# Autodesk Inventor assembly: Drive Roller Assembly 2
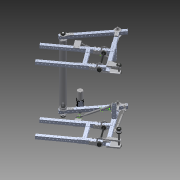
[picture p0: Inventor's stored thumbnail of the model, 180x180]
Saved by Autodesk Inventor 2014 (Build 180170000, 170)
## iProperties
Created: 2014-01-12
Part Number: Drive Roller Assembly 2
Document SubType Name: Assembly
Designer: Michael
Mass: 4835.9 g
Surface Area: 14934.6 cm^2
Volume: 1370.56 cm^3
Density: 3.52842 g/cm^3
Author: Michael
## Documents named in this file (35)
- C:\Users\Michael\Documents\GitHub\2014buildCAD\New Collector\Drive Roller Assembly 2.iam
- C:\Users\Michael\Documents\GitHub\2014buildCAD\Collector\Hex Shaft Collar 1-2 in (7552K500).ipt
- C:\Users\Michael\Documents\GitHub\2014buildCAD\Collector\Roller End Cap Drive (3-D Printed).ipt
- C:\Users\Michael\Documents\GitHub\2014buildCAD\Collector\Vex Pro VersaPlanetary Side Mount.ipt
- C:\Users\Michael\Documents\GitHub\2014buildCAD\Collector\VersaPlanetary (Fixed).iam
- C:\Users\Michael\Documents\GitHub\2014buildCAD\New Collector\Polycarbonate Roller 2 OD 1-16 Thick (8585K64).ipt
- C:\Users\Michael\Documents\GitHub\2014buildCAD\New Collector\Hex Bearing 1-2 in (FR8ZZ-Hex, am-0279).ipt
- C:\Users\Michael\Documents\GitHub\2014buildCAD\New Collector\Hex Shaft Collar 1-2 in (7552K500).ipt
- C:\Users\Michael\Documents\GitHub\2014buildCAD\New Collector\Roller End Cap Drive (3-D Printed).ipt
- C:\Users\Michael\Documents\GitHub\2014buildCAD\New Collector\Vex Pro End Bearing Mount.ipt
- C:\Users\Michael\Documents\GitHub\2014buildCAD\New Collector\Vex Pro 1x1 rectangular tubing 14 in length.ipt
- C:\Users\Michael\Documents\GitHub\2014buildCAD\New Collector\Hex Shaft Aluminum 1-2 in (am-2291).ipt
- C:\Users\Michael\Documents\GitHub\2014buildCAD\New Collector\Timing Pulley (HTD 5mm) - 18T 9mm Double Flange, 1-2 in Hex (VexPro).ipt
- C:\Users\Michael\Documents\GitHub\2014buildCAD\New Collector\Clamp with Piston Assembly.iam
- C:\Users\Michael\Documents\GitHub\2014buildCAD\New Collector\Vex Pro 90 degree gusset.ipt
- C:\Users\Michael\Documents\GitHub\2014buildCAD\New Collector\Vex Pro 1x1 rectangular tubing 2 in length.ipt
- C:\Users\Michael\Documents\GitHub\2014buildCAD\New Collector\Hex Shaft 3-8 in (am-0855).ipt
- C:\Users\Michael\Documents\GitHub\2014buildCAD\New Collector\Hex Shaft Collar 3-8 in (7552K300).ipt
- C:\Users\Michael\Documents\GitHub\2014buildCAD\New Collector\3 Postion Pneumatic Cylinder (9-16 in Bore, .25 in,2 in stroke).iam
- C:\Users\Michael\Documents\GitHub\2014buildCAD\New Collector\Hex Shaft 1-2 in (am-0856).ipt
- C:\Users\Michael\Documents\GitHub\2014buildCAD\New Collector\Spacer 2.ipt
- C:\Users\Michael\Documents\GitHub\2014buildCAD\New Collector\Gusset 3 (R-R) (Custom) ipt.ipt
- C:\Users\Michael\Documents\GitHub\2014buildCAD\New Collector\Gusset 3 (L-R) (Custom).ipt
- C:\Users\Michael\Documents\GitHub\2014buildCAD\New Collector\Gusset 3 (L-L) (Custom) ipt.ipt
- C:\Users\Michael\Documents\GitHub\2014buildCAD\New Collector\Gusset 3 (R-L) (Custom).ipt
- C:\Users\Michael\Documents\GitHub\2014buildCAD\New Collector\Vex Pro 1x1 rectangular tubing 4 in length.ipt
- C:\Users\Michael\Documents\GitHub\2014buildCAD\New Collector\Pneumatic Piston Front Flange (Lt Custom).ipt
- C:\Users\Michael\Documents\GitHub\2014buildCAD\New Collector\Pneumatic Piston Front Flange (Rt Custom).ipt
- C:\Users\Michael\Documents\GitHub\2014buildCAD\New Collector\Pneumatic Piston Back Flange (Rt Custom).ipt
- C:\Users\Michael\Documents\GitHub\2014buildCAD\New Collector\Bearing Mount Spacer 1-8 in.ipt
- C:\Users\Michael\Documents\GitHub\2014buildCAD\New Collector\Vex Pro 1x1 rectangular tubing 14 in length (roller).ipt
- C:\Users\Michael\Documents\GitHub\2014buildCAD\New Collector\Pneumatic Piston Back Flange (Right Custom).ipt
- C:\Users\Michael\Documents\GitHub\2014buildCAD\New Collector\Hex Shaft 1-2 in 5 in long (am-0856).ipt
- C:\Users\Michael\Documents\GitHub\2014buildCAD\New Collector\Vex Pro End Bearing Mount (Bolt).ipt
- C:\Users\Michael\Documents\GitHub\2014buildCAD\New Collector\Roller Piston (3 Position, .25 and 1.125 in stroke, 9-16 bore).iam
## Components (96 placed, 32 different names)
1. Roller End Cap Drive (3-D Printed):2 — Mate:154, Mate:155, Mate:157, Mate:158, Mate:466, Mate:469
2. Vex Pro VersaPlanetary Side Mount:1 — Insert:29, Insert:30, Mate:566, Mate:779, Mate:780
3. VersaPlanetary (Fixed):1 [sub-assembly] — Insert:29, Insert:30, Mate:113, Mate:114, Mate:120, Mate:121, Mate:153
4. Hex Shaft Collar 1-2 in (7552K500):9 — Mate:113, Mate:114
5. Hex Shaft Collar 1-2 in (7552K500):10 — Mate:120, Mate:121
6. Polycarbonate Roller 2 OD 1-16 Thick (8585K64):3 — Mate:157, Mate:158, Mate:159, Mate:160
7. Hex Bearing 1-2 in (FR8ZZ-Hex, am-0279):3 — Mate:128, Mate:129, Mate:134, Mate:466
8. Roller End Cap Drive (3-D Printed):5 — Mate:159, Mate:160, Mate:632, Mate:635
9. Hex Shaft Aluminum 1-2 in (am-2291):1 — Flush:1, Mate:132, Mate:133, Mate:134, Mate:143, Mate:144, Mate:146, Mate:147, Mate:154, Mate:155, Mate:172, Mate:173, Mate:179, Mate:180, Mate:467, Mate:468
10. Vex Pro End Bearing Mount:4 — Mate:130, Mate:131, Mate:621, Mate:764, Mate:765
11. Vex Pro End Bearing Mount:5 — Mate:128, Mate:129, Mate:624, Mate:762, Mate:763
12. Hex Bearing 1-2 in (FR8ZZ-Hex, am-0279):4 — Mate:130, Mate:131, Flush:1, Mate:132, Mate:133, Mate:161
13. Timing Pulley (HTD 5mm) - 18T 9mm Double Flange, 1-2 in Hex (VexPro):3 — Mate:143, Mate:144, Mate:145, Mate:161
14. Hex Shaft Collar 1-2 in (7552K500):13 — Mate:145, Mate:146, Mate:147, Flush:2
15. Hex Shaft Collar 1-2 in (7552K500):14 — Flush:4, Mate:152
16. Timing Pulley (HTD 5mm) - 18T 9mm Double Flange, 1-2 in Hex (VexPro):4 — Mate:150, Flush:3, Mate:151, Flush:4, Mate:152
17. Hex Shaft Collar 1-2 in (7552K500):15 — Flush:2, Mate:150, Flush:3, Mate:151, Mate:153
18. Hex Bearing 1-2 in (FR8ZZ-Hex, am-0279):5 — Mate:178, Mate:758, Mate:759
19. Vex Pro End Bearing Mount:7 — Mate:631, Mate:766, Mate:767
20. Vex Pro End Bearing Mount:8 — Mate:629, Mate:760, Mate:761
21. Hex Bearing 1-2 in (FR8ZZ-Hex, am-0279):6 — Mate:172, Mate:173, Mate:470, Mate:471, Mate:632
22. Hex Shaft Collar 1-2 in (7552K500):16 — Mate:178, Mate:179, Mate:180, Flush:13
23. Clamp with Piston Assembly:1 [sub-assembly] — Mate:226, Mate:227, Flush:6, Mate:230, Mate:233, Mate:673, Mate:689, Mate:690
24. Vex Pro 1x1 rectangular tubing 14 in length:5 — Mate:203, Mate:210, Mate:211, Mate:221, Mate:222, Mate:223, Mate:326, Mate:328, Mate:329, Mate:427, Mate:429, Mate:615, Mate:618, Flush:20, Mate:653, Mate:654, Mate:655, Flush:24, Flush:25
25. Vex Pro 1x1 rectangular tubing 14 in length:6 — Mate:258, Mate:259, Mate:260, Mate:263, Mate:320, Mate:321, Mate:322, Mate:323, Mate:418, Mate:419, Mate:420, Mate:546, Mate:555, Flush:20, Mate:642, Mate:658, Mate:660, Mate:661, Mate:776, Mate:777, Mate:778, Mate:788, Mate:789
26. Vex Pro 90 degree gusset:8 — Mate:203, Mate:210, Mate:211, Mate:212, Mate:213, Mate:214
27. Vex Pro 1x1 rectangular tubing 2 in length:1 — Mate:212, Mate:213, Mate:214, Mate:327
28. Vex Pro 90 degree gusset:10 — Mate:221, Mate:222, Mate:223, Mate:433, Mate:434, Mate:435
29. Vex Pro 1x1 rectangular tubing 2 in length:2 — Mate:224, Mate:225, Flush:5, Mate:428
30. Hex Shaft 3-8 in (am-0855):1 — Mate:224, Mate:225, Flush:5, Mate:226, Mate:227, Flush:6, Mate:228, Mate:229, Mate:231, Mate:232
31. Hex Shaft Collar 3-8 in (7552K300):1 — Mate:228, Mate:229, Mate:230
32. Hex Shaft Collar 3-8 in (7552K300):2 — Mate:231, Mate:232, Mate:233
33. Clamp with Piston Assembly:2 [sub-assembly] — Mate:666, Mate:668, Mate:669
34. Vex Pro 90 degree gusset:11 — Mate:322, Mate:323, Mate:642
35. Vex Pro 90 degree gusset:12 — Mate:263, Mate:320, Mate:321, Mate:324, Mate:325
36. Vex Pro 1x1 rectangular tubing 2 in length:3 — Mate:324, Mate:325
37. Vex Pro 90 degree gusset:13 — Mate:258, Mate:259, Mate:260, Mate:425, Mate:426, Mate:492
38. Vex Pro 1x1 rectangular tubing 2 in length:4
39. Hex Shaft 3-8 in (am-0855):2
40. Hex Shaft Collar 3-8 in (7552K300):3
41. Hex Shaft Collar 3-8 in (7552K300):4
42. 3 Postion Pneumatic Cylinder (9-16 in Bore, .25 in,2 in stroke):1 [sub-assembly] — Mate:686, Mate:687, Mate:688, Mate:691
43. Vex Pro 90 degree gusset:14 — Mate:476, Mate:477, Mate:478, Mate:653, Mate:654, Mate:655
44. Vex Pro 90 degree gusset:15 — Mate:650, Mate:651, Mate:652
45. Vex Pro 90 degree gusset:17 — Mate:485, Mate:486, Mate:487
46. Vex Pro 90 degree gusset:18 — Mate:656, Mate:657, Mate:658, Mate:659, Mate:660, Mate:661, Mate:783
47. Vex Pro 90 degree gusset:19 — Mate:326, Mate:327, Mate:328, Mate:329
48. Hex Shaft 1-2 in (am-0856):2 — Mate:402, Mate:403, Mate:405, Mate:406, Mate:447, Mate:448, Flush:12
49. Hex Shaft Collar 1-2 in (7552K500):18 — Mate:402, Mate:403, Mate:450, Flush:12
50. Hex Shaft Collar 1-2 in (7552K500):19 — Mate:405, Mate:406, Mate:449
51. Hex Shaft Collar 1-2 in (7552K500):20 — Mate:706, Mate:707, Mate:712, Mate:726
52. Hex Shaft Collar 1-2 in (7552K500):21 — Mate:446, Mate:704, Mate:705, Flush:22
53. Spacer 2:1 — Mate:418, Mate:419, Mate:420, Mate:438, Mate:439, Mate:451, Mate:452, Mate:453
54. Gusset 3 (R-R) (Custom) ipt:1 — Mate:425, Mate:426, Mate:446, Mate:492
55. Spacer 2:2 — Mate:427, Mate:428, Mate:429, Mate:430, Mate:431, Mate:455, Mate:456, Mate:457
56. Gusset 3 (L-R) (Custom):1 — Mate:430, Mate:431, Mate:447, Mate:448, Mate:450, Mate:461
57. Gusset 3 (L-L) (Custom) ipt:1 — Mate:433, Mate:434, Mate:435, Mate:449
58. Gusset 3 (R-L) (Custom):1 — Mate:438, Mate:439, Mate:465, Mate:708, Mate:709, Mate:726
59. Spacer 2:3 — Mate:451, Mate:452, Mate:453, Mate:462, Mate:463, Mate:464
60. Spacer 2:4 — Mate:455, Mate:456, Mate:457, Mate:458, Mate:459, Mate:460
61. Spacer 2:5 — Mate:458, Mate:459, Mate:460, Mate:461
62. Spacer 2:6 — Mate:462, Mate:463, Mate:464, Mate:465
63. Hex Shaft Collar 1-2 in (7552K500):22 — Mate:467, Mate:468, Mate:469
64. Hex Shaft Aluminum 1-2 in (am-2291):2 — Mate:470, Mate:471, Flush:13, Mate:633, Mate:634, Mate:758, Mate:759
65. Vex Pro 1x1 rectangular tubing 4 in length:1 — Mate:476, Mate:477, Mate:478, Mate:650, Mate:651, Mate:652, Mate:683, Mate:684, Mate:685
66. Vex Pro 1x1 rectangular tubing 4 in length:2 — Mate:485, Mate:486, Mate:487, Mate:656, Mate:657, Mate:659, Mate:694, Mate:699, Mate:700
67. 3 Postion Pneumatic Cylinder (9-16 in Bore, .25 in,2 in stroke):2 [sub-assembly] — Mate:701, Mate:702, Mate:703, Mate:751
68. Bearing Mount Spacer 1-8 in:1 — Mate:748, Mate:749, Mate:750
69. Bearing Mount Spacer 1-8 in:2 — Mate:546, Mate:776, Mate:777
70. Bearing Mount Spacer 1-8 in:3 — Mate:743, Mate:744, Mate:745
71. Bearing Mount Spacer 1-8 in:4 — Mate:555, Mate:778
72. Hex Bearing 1-2 in (FR8ZZ-Hex, am-0279):7 — Flush:15, Mate:560, Mate:561, Mate:567, Flush:23, Mate:754, Mate:755
73. Hex Shaft 1-2 in (am-0856):4 — Mate:560, Mate:561, Mate:562, Mate:563, Flush:23, Mate:774
74. Hex Bearing 1-2 in (FR8ZZ-Hex, am-0279):8 — Flush:15, Mate:746, Mate:747, Mate:774
75. Vex Pro 1x1 rectangular tubing 14 in length (roller):1 — Mate:562, Mate:563, Mate:566, Mate:567, Mate:621, Mate:624, Flush:21, Mate:762, Mate:763, Mate:764, Mate:765, Mate:779, Mate:780, Angle:1
76. Bearing Mount Spacer 1-8 in:5 — Mate:740, Mate:741, Mate:742
77. Bearing Mount Spacer 1-8 in:6 — Mate:618
78. Bearing Mount Spacer 1-8 in:7 — Mate:735, Mate:736, Mate:737
79. Bearing Mount Spacer 1-8 in:8 — Mate:615, Flush:24
80. Hex Bearing 1-2 in (FR8ZZ-Hex, am-0279):9 — Flush:19, Mate:752, Mate:753
81. Hex Shaft 1-2 in (am-0856):5 — Flush:19, Mate:775
82. Hex Bearing 1-2 in (FR8ZZ-Hex, am-0279):10 — Mate:738, Mate:739, Mate:775
83. Vex Pro 1x1 rectangular tubing 14 in length (roller):2 — Mate:629, Mate:631, Flush:21, Mate:760, Mate:761, Mate:766, Mate:767
84. Hex Shaft Collar 1-2 in (7552K500):23 — Mate:633, Mate:634, Mate:635
85. Pneumatic Piston Front Flange (Rt Custom):2 — Mate:666, Mate:668, Mate:669, Mate:751
86. Pneumatic Piston Front Flange (Lt Custom):1 — Mate:673, Mate:689, Mate:690, Mate:691
87. Pneumatic Piston Back Flange (Rt Custom):1 — Mate:683, Mate:684, Mate:685, Mate:686, Mate:687, Mate:688
88. Pneumatic Piston Back Flange (Right Custom):1 — Mate:694, Mate:699, Mate:700, Mate:701, Mate:702, Mate:703
89. Hex Shaft 1-2 in 5 in long (am-0856):1 — Mate:704, Mate:705, Mate:706, Mate:707, Mate:708, Mate:709, Flush:22, Mate:710, Mate:711, Mate:714, Mate:715
90. Timing Pulley (HTD 5mm) - 18T 9mm Double Flange, 1-2 in Hex (VexPro):5 — Mate:710, Mate:711, Mate:712, Mate:713
91. Hex Shaft Collar 1-2 in (7552K500):24 — Mate:713, Mate:714, Mate:715
92. Vex Pro End Bearing Mount (Bolt):1 — Mate:735, Mate:736, Mate:737, Mate:738, Mate:739
93. Vex Pro End Bearing Mount (Bolt):2 — Mate:740, Mate:741, Mate:742, Mate:752, Mate:753, Flush:25
94. Vex Pro End Bearing Mount (Bolt):3 — Mate:743, Mate:744, Mate:745, Mate:746, Mate:747
95. Vex Pro End Bearing Mount (Bolt):4 — Mate:748, Mate:749, Mate:750, Mate:754, Mate:755
96. Roller Piston (3 Position, .25 and 1.125 in stroke, 9-16 bore):1 [sub-assembly] — Mate:783, Mate:788, Mate:789, Angle:1
## Relationships (282: Mate 260, Flush 19, Insert 2, Angle 1)
- Insert:29: Vex Pro VersaPlanetary Side Mount:1 ↔ VersaPlanetary (Fixed):1
- Insert:30: Vex Pro VersaPlanetary Side Mount:1 ↔ VersaPlanetary (Fixed):1
- Mate:113: VersaPlanetary (Fixed):1 ↔ Hex Shaft Collar 1-2 in (7552K500):9
- Mate:114: VersaPlanetary (Fixed):1 ↔ Hex Shaft Collar 1-2 in (7552K500):9
- Mate:120: VersaPlanetary (Fixed):1 ↔ Hex Shaft Collar 1-2 in (7552K500):10
- Mate:121: VersaPlanetary (Fixed):1 ↔ Hex Shaft Collar 1-2 in (7552K500):10
- Mate:128: Hex Bearing 1-2 in (FR8ZZ-Hex, am-0279):3 ↔ Vex Pro End Bearing Mount:5
- Mate:129: Hex Bearing 1-2 in (FR8ZZ-Hex, am-0279):3 ↔ Vex Pro End Bearing Mount:5
- Mate:130: Vex Pro End Bearing Mount:4 ↔ Hex Bearing 1-2 in (FR8ZZ-Hex, am-0279):4
- Mate:131: Vex Pro End Bearing Mount:4 ↔ Hex Bearing 1-2 in (FR8ZZ-Hex, am-0279):4
- Flush:1 (-25.4 mm): Hex Shaft Aluminum 1-2 in (am-2291):1 ↔ Hex Bearing 1-2 in (FR8ZZ-Hex, am-0279):4
- Mate:132: Hex Shaft Aluminum 1-2 in (am-2291):1 ↔ Hex Bearing 1-2 in (FR8ZZ-Hex, am-0279):4
- Mate:133: Hex Shaft Aluminum 1-2 in (am-2291):1 ↔ Hex Bearing 1-2 in (FR8ZZ-Hex, am-0279):4
- Mate:134: Hex Bearing 1-2 in (FR8ZZ-Hex, am-0279):3 ↔ Hex Shaft Aluminum 1-2 in (am-2291):1
- Mate:143: Hex Shaft Aluminum 1-2 in (am-2291):1 ↔ Timing Pulley (HTD 5mm) - 18T 9mm Double Flange, 1-2 in Hex (VexPro):3
- Mate:144: Hex Shaft Aluminum 1-2 in (am-2291):1 ↔ Timing Pulley (HTD 5mm) - 18T 9mm Double Flange, 1-2 in Hex (VexPro):3
- Mate:145: Timing Pulley (HTD 5mm) - 18T 9mm Double Flange, 1-2 in Hex (VexPro):3 ↔ Hex Shaft Collar 1-2 in (7552K500):13
- Mate:146: Hex Shaft Aluminum 1-2 in (am-2291):1 ↔ Hex Shaft Collar 1-2 in (7552K500):13
- Mate:147: Hex Shaft Aluminum 1-2 in (am-2291):1 ↔ Hex Shaft Collar 1-2 in (7552K500):13
- [Mate]: Hex Shaft Collar 1-2 in (7552K500):14 ↔ Timing Pulley (HTD 5mm) - 18T 9mm Double Flange, 1-2 in Hex (VexPro):4
- [Mate]: Timing Pulley (HTD 5mm) - 18T 9mm Double Flange, 1-2 in Hex (VexPro):4 ↔ Hex Shaft Collar 1-2 in (7552K500):15
- Flush:2: Hex Shaft Collar 1-2 in (7552K500):13 ↔ Hex Shaft Collar 1-2 in (7552K500):15
- Mate:150: Timing Pulley (HTD 5mm) - 18T 9mm Double Flange, 1-2 in Hex (VexPro):4 ↔ Hex Shaft Collar 1-2 in (7552K500):15
- Flush:3: Timing Pulley (HTD 5mm) - 18T 9mm Double Flange, 1-2 in Hex (VexPro):4 ↔ Hex Shaft Collar 1-2 in (7552K500):15
- Mate:151: Timing Pulley (HTD 5mm) - 18T 9mm Double Flange, 1-2 in Hex (VexPro):4 ↔ Hex Shaft Collar 1-2 in (7552K500):15
- Flush:4: Hex Shaft Collar 1-2 in (7552K500):14 ↔ Timing Pulley (HTD 5mm) - 18T 9mm Double Flange, 1-2 in Hex (VexPro):4
- Mate:152: Hex Shaft Collar 1-2 in (7552K500):14 ↔ Timing Pulley (HTD 5mm) - 18T 9mm Double Flange, 1-2 in Hex (VexPro):4
- Mate:153: VersaPlanetary (Fixed):1 ↔ Hex Shaft Collar 1-2 in (7552K500):15
- Mate:154: Roller End Cap Drive (3-D Printed):2 ↔ Hex Shaft Aluminum 1-2 in (am-2291):1
- Mate:155: Roller End Cap Drive (3-D Printed):2 ↔ Hex Shaft Aluminum 1-2 in (am-2291):1
- Mate:157: Roller End Cap Drive (3-D Printed):2 ↔ Polycarbonate Roller 2 OD 1-16 Thick (8585K64):3
- Mate:158: Roller End Cap Drive (3-D Printed):2 ↔ Polycarbonate Roller 2 OD 1-16 Thick (8585K64):3
- Mate:159: Polycarbonate Roller 2 OD 1-16 Thick (8585K64):3 ↔ Roller End Cap Drive (3-D Printed):5
- Mate:160: Polycarbonate Roller 2 OD 1-16 Thick (8585K64):3 ↔ Roller End Cap Drive (3-D Printed):5
- Mate:161: Hex Bearing 1-2 in (FR8ZZ-Hex, am-0279):4 ↔ Timing Pulley (HTD 5mm) - 18T 9mm Double Flange, 1-2 in Hex (VexPro):3
- [Mate]: Hex Bearing 1-2 in (FR8ZZ-Hex, am-0279):5 ↔ Vex Pro End Bearing Mount:8
- [Mate]: Hex Bearing 1-2 in (FR8ZZ-Hex, am-0279):5 ↔ Vex Pro End Bearing Mount:8
- [Mate]: Vex Pro End Bearing Mount:7 ↔ Hex Bearing 1-2 in (FR8ZZ-Hex, am-0279):6
- [Mate]: Vex Pro End Bearing Mount:7 ↔ Hex Bearing 1-2 in (FR8ZZ-Hex, am-0279):6
- Mate:172: Hex Shaft Aluminum 1-2 in (am-2291):1 ↔ Hex Bearing 1-2 in (FR8ZZ-Hex, am-0279):6
- Mate:173: Hex Shaft Aluminum 1-2 in (am-2291):1 ↔ Hex Bearing 1-2 in (FR8ZZ-Hex, am-0279):6
- Mate:178: Hex Bearing 1-2 in (FR8ZZ-Hex, am-0279):5 ↔ Hex Shaft Collar 1-2 in (7552K500):16
- Mate:179: Hex Shaft Aluminum 1-2 in (am-2291):1 ↔ Hex Shaft Collar 1-2 in (7552K500):16
- Mate:180: Hex Shaft Aluminum 1-2 in (am-2291):1 ↔ Hex Shaft Collar 1-2 in (7552K500):16
- Mate:203: Vex Pro 1x1 rectangular tubing 14 in length:5 ↔ Vex Pro 90 degree gusset:8
- Mate:210: Vex Pro 1x1 rectangular tubing 14 in length:5 ↔ Vex Pro 90 degree gusset:8
- Mate:211: Vex Pro 1x1 rectangular tubing 14 in length:5 ↔ Vex Pro 90 degree gusset:8
- Mate:212: Vex Pro 90 degree gusset:8 ↔ Vex Pro 1x1 rectangular tubing 2 in length:1
- Mate:213: Vex Pro 90 degree gusset:8 ↔ Vex Pro 1x1 rectangular tubing 2 in length:1
- Mate:214: Vex Pro 90 degree gusset:8 ↔ Vex Pro 1x1 rectangular tubing 2 in length:1
- [Mate]: Vex Pro 90 degree gusset:10 ↔ Vex Pro 1x1 rectangular tubing 2 in length:2
- [Mate]: Vex Pro 90 degree gusset:10 ↔ Vex Pro 1x1 rectangular tubing 2 in length:2
- [Mate]: Vex Pro 90 degree gusset:10 ↔ Vex Pro 1x1 rectangular tubing 2 in length:2
- Mate:221: Vex Pro 1x1 rectangular tubing 14 in length:5 ↔ Vex Pro 90 degree gusset:10
- Mate:222: Vex Pro 1x1 rectangular tubing 14 in length:5 ↔ Vex Pro 90 degree gusset:10
- Mate:223: Vex Pro 1x1 rectangular tubing 14 in length:5 ↔ Vex Pro 90 degree gusset:10
- Mate:224: Vex Pro 1x1 rectangular tubing 2 in length:2 ↔ Hex Shaft 3-8 in (am-0855):1
- Mate:225: Vex Pro 1x1 rectangular tubing 2 in length:2 ↔ Hex Shaft 3-8 in (am-0855):1
- Flush:5 (-19.05 mm): Vex Pro 1x1 rectangular tubing 2 in length:2 ↔ Hex Shaft 3-8 in (am-0855):1
- Mate:226: Clamp with Piston Assembly:1 ↔ Hex Shaft 3-8 in (am-0855):1
- Mate:227: Clamp with Piston Assembly:1 ↔ Hex Shaft 3-8 in (am-0855):1
- Flush:6 (-9.525 mm): Clamp with Piston Assembly:1 ↔ Hex Shaft 3-8 in (am-0855):1
- Mate:228: Hex Shaft 3-8 in (am-0855):1 ↔ Hex Shaft Collar 3-8 in (7552K300):1
- Mate:229: Hex Shaft 3-8 in (am-0855):1 ↔ Hex Shaft Collar 3-8 in (7552K300):1
- Mate:230: Clamp with Piston Assembly:1 ↔ Hex Shaft Collar 3-8 in (7552K300):1
- Mate:231: Hex Shaft 3-8 in (am-0855):1 ↔ Hex Shaft Collar 3-8 in (7552K300):2
- Mate:232: Hex Shaft 3-8 in (am-0855):1 ↔ Hex Shaft Collar 3-8 in (7552K300):2
- Mate:233: Clamp with Piston Assembly:1 ↔ Hex Shaft Collar 3-8 in (7552K300):2
- [Mate]: Vex Pro 90 degree gusset:12 ↔ Vex Pro 1x1 rectangular tubing 2 in length:3
- [Mate]: Vex Pro 90 degree gusset:13 ↔ Vex Pro 1x1 rectangular tubing 2 in length:4
- [Mate]: Vex Pro 90 degree gusset:13 ↔ Vex Pro 1x1 rectangular tubing 2 in length:4
- [Mate]: Vex Pro 90 degree gusset:13 ↔ Vex Pro 1x1 rectangular tubing 2 in length:4
- [Mate]: Vex Pro 1x1 rectangular tubing 2 in length:4 ↔ Hex Shaft 3-8 in (am-0855):2
- [Mate]: Vex Pro 1x1 rectangular tubing 2 in length:4 ↔ Hex Shaft 3-8 in (am-0855):2
- [Flush] (-19.05 mm): Vex Pro 1x1 rectangular tubing 2 in length:4 ↔ Hex Shaft 3-8 in (am-0855):2
- [Mate]: Clamp with Piston Assembly:2 ↔ Hex Shaft 3-8 in (am-0855):2
- [Mate]: Clamp with Piston Assembly:2 ↔ Hex Shaft 3-8 in (am-0855):2
- [Flush] (-9.525 mm): Clamp with Piston Assembly:2 ↔ Hex Shaft 3-8 in (am-0855):2
- [Mate]: Hex Shaft 3-8 in (am-0855):2 ↔ Hex Shaft Collar 3-8 in (7552K300):3
- [Mate]: Hex Shaft 3-8 in (am-0855):2 ↔ Hex Shaft Collar 3-8 in (7552K300):3
- [Mate]: Clamp with Piston Assembly:2 ↔ Hex Shaft Collar 3-8 in (7552K300):3
- [Mate]: Hex Shaft 3-8 in (am-0855):2 ↔ Hex Shaft Collar 3-8 in (7552K300):4
- [Mate]: Hex Shaft 3-8 in (am-0855):2 ↔ Hex Shaft Collar 3-8 in (7552K300):4
- [Mate]: Clamp with Piston Assembly:2 ↔ Hex Shaft Collar 3-8 in (7552K300):4
- Mate:258: Vex Pro 1x1 rectangular tubing 14 in length:6 ↔ Vex Pro 90 degree gusset:13
- Mate:259: Vex Pro 1x1 rectangular tubing 14 in length:6 ↔ Vex Pro 90 degree gusset:13
- Mate:260: Vex Pro 1x1 rectangular tubing 14 in length:6 ↔ Vex Pro 90 degree gusset:13
- Mate:263: Vex Pro 1x1 rectangular tubing 14 in length:6 ↔ Vex Pro 90 degree gusset:12
- Mate:320: Vex Pro 1x1 rectangular tubing 14 in length:6 ↔ Vex Pro 90 degree gusset:12
- Mate:321: Vex Pro 1x1 rectangular tubing 14 in length:6 ↔ Vex Pro 90 degree gusset:12
- Mate:322: Vex Pro 1x1 rectangular tubing 14 in length:6 ↔ Vex Pro 90 degree gusset:11
- Mate:323: Vex Pro 1x1 rectangular tubing 14 in length:6 ↔ Vex Pro 90 degree gusset:11
- Mate:324: Vex Pro 90 degree gusset:12 ↔ Vex Pro 1x1 rectangular tubing 2 in length:3
- Mate:325: Vex Pro 90 degree gusset:12 ↔ Vex Pro 1x1 rectangular tubing 2 in length:3
- Mate:326: Vex Pro 1x1 rectangular tubing 14 in length:5 ↔ Vex Pro 90 degree gusset:19
- Mate:327: Vex Pro 1x1 rectangular tubing 2 in length:1 ↔ Vex Pro 90 degree gusset:19
- Mate:328: Vex Pro 1x1 rectangular tubing 14 in length:5 ↔ Vex Pro 90 degree gusset:19
- Mate:329: Vex Pro 1x1 rectangular tubing 14 in length:5 ↔ Vex Pro 90 degree gusset:19
- Mate:402: Hex Shaft 1-2 in (am-0856):2 ↔ Hex Shaft Collar 1-2 in (7552K500):18
- Mate:403: Hex Shaft 1-2 in (am-0856):2 ↔ Hex Shaft Collar 1-2 in (7552K500):18
- Mate:405: Hex Shaft 1-2 in (am-0856):2 ↔ Hex Shaft Collar 1-2 in (7552K500):19
- Mate:406: Hex Shaft 1-2 in (am-0856):2 ↔ Hex Shaft Collar 1-2 in (7552K500):19
- Mate:418: Vex Pro 1x1 rectangular tubing 14 in length:6 ↔ Spacer 2:1
- Mate:419: Vex Pro 1x1 rectangular tubing 14 in length:6 ↔ Spacer 2:1
- Mate:420: Vex Pro 1x1 rectangular tubing 14 in length:6 ↔ Spacer 2:1
- Mate:425: Vex Pro 90 degree gusset:13 ↔ Gusset 3 (R-R) (Custom) ipt:1
- Mate:426: Vex Pro 90 degree gusset:13 ↔ Gusset 3 (R-R) (Custom) ipt:1
- Mate:427: Vex Pro 1x1 rectangular tubing 14 in length:5 ↔ Spacer 2:2
- Mate:428: Vex Pro 1x1 rectangular tubing 2 in length:2 ↔ Spacer 2:2
- Mate:429: Vex Pro 1x1 rectangular tubing 14 in length:5 ↔ Spacer 2:2
- Mate:430: Spacer 2:2 ↔ Gusset 3 (L-R) (Custom):1
- Mate:431: Spacer 2:2 ↔ Gusset 3 (L-R) (Custom):1
- Mate:433: Vex Pro 90 degree gusset:10 ↔ Gusset 3 (L-L) (Custom) ipt:1
- Mate:434: Vex Pro 90 degree gusset:10 ↔ Gusset 3 (L-L) (Custom) ipt:1
- Mate:435: Vex Pro 90 degree gusset:10 ↔ Gusset 3 (L-L) (Custom) ipt:1
- Mate:438: Spacer 2:1 ↔ Gusset 3 (R-L) (Custom):1
- Mate:439: Spacer 2:1 ↔ Gusset 3 (R-L) (Custom):1
- Mate:446: Hex Shaft Collar 1-2 in (7552K500):21 ↔ Gusset 3 (R-R) (Custom) ipt:1
- Mate:447: Hex Shaft 1-2 in (am-0856):2 ↔ Gusset 3 (L-R) (Custom):1
- Mate:448: Hex Shaft 1-2 in (am-0856):2 ↔ Gusset 3 (L-R) (Custom):1
- Mate:449: Hex Shaft Collar 1-2 in (7552K500):19 ↔ Gusset 3 (L-L) (Custom) ipt:1
- Mate:450: Hex Shaft Collar 1-2 in (7552K500):18 ↔ Gusset 3 (L-R) (Custom):1
- Mate:451: Spacer 2:1 ↔ Spacer 2:3
- Mate:452: Spacer 2:1 ↔ Spacer 2:3
- Mate:453: Spacer 2:1 ↔ Spacer 2:3
- Mate:455: Spacer 2:2 ↔ Spacer 2:4
- Mate:456: Spacer 2:2 ↔ Spacer 2:4
- Mate:457: Spacer 2:2 ↔ Spacer 2:4
- Mate:458: Spacer 2:4 ↔ Spacer 2:5
- Mate:459: Spacer 2:4 ↔ Spacer 2:5
- Mate:460: Spacer 2:4 ↔ Spacer 2:5
- Mate:461: Gusset 3 (L-R) (Custom):1 ↔ Spacer 2:5
- Mate:462: Spacer 2:3 ↔ Spacer 2:6
- Mate:463: Spacer 2:3 ↔ Spacer 2:6
- Mate:464: Spacer 2:3 ↔ Spacer 2:6
- Mate:465: Gusset 3 (R-L) (Custom):1 ↔ Spacer 2:6
- Flush:12 (-9.525 mm): Hex Shaft 1-2 in (am-0856):2 ↔ Hex Shaft Collar 1-2 in (7552K500):18
- Mate:466: Roller End Cap Drive (3-D Printed):2 ↔ Hex Bearing 1-2 in (FR8ZZ-Hex, am-0279):3
- Mate:467: Hex Shaft Aluminum 1-2 in (am-2291):1 ↔ Hex Shaft Collar 1-2 in (7552K500):22
- Mate:468: Hex Shaft Aluminum 1-2 in (am-2291):1 ↔ Hex Shaft Collar 1-2 in (7552K500):22
- Mate:469: Roller End Cap Drive (3-D Printed):2 ↔ Hex Shaft Collar 1-2 in (7552K500):22
- Mate:470: Hex Bearing 1-2 in (FR8ZZ-Hex, am-0279):6 ↔ Hex Shaft Aluminum 1-2 in (am-2291):2
- Mate:471: Hex Bearing 1-2 in (FR8ZZ-Hex, am-0279):6 ↔ Hex Shaft Aluminum 1-2 in (am-2291):2
- Flush:13 (-3.175 mm): Hex Shaft Collar 1-2 in (7552K500):16 ↔ Hex Shaft Aluminum 1-2 in (am-2291):2
- Mate:476: Vex Pro 90 degree gusset:14 ↔ Vex Pro 1x1 rectangular tubing 4 in length:1
- Mate:477: Vex Pro 90 degree gusset:14 ↔ Vex Pro 1x1 rectangular tubing 4 in length:1
- Mate:478: Vex Pro 90 degree gusset:14 ↔ Vex Pro 1x1 rectangular tubing 4 in length:1
- Mate:485: Vex Pro 90 degree gusset:17 ↔ Vex Pro 1x1 rectangular tubing 4 in length:2
- Mate:486: Vex Pro 90 degree gusset:17 ↔ Vex Pro 1x1 rectangular tubing 4 in length:2
- Mate:487: Vex Pro 90 degree gusset:17 ↔ Vex Pro 1x1 rectangular tubing 4 in length:2
- Mate:492: Vex Pro 90 degree gusset:13 ↔ Gusset 3 (R-R) (Custom) ipt:1
- [Mate]: Bearing Mount Spacer 1-8 in:1 ↔ Bearing Mount Spacer 1-8 in:2
- [Mate]: Bearing Mount Spacer 1-8 in:1 ↔ Bearing Mount Spacer 1-8 in:2
- [Mate]: Bearing Mount Spacer 1-8 in:1 ↔ Bearing Mount Spacer 1-8 in:2
- Mate:546: Vex Pro 1x1 rectangular tubing 14 in length:6 ↔ Bearing Mount Spacer 1-8 in:2
- [Mate]: Bearing Mount Spacer 1-8 in:3 ↔ Bearing Mount Spacer 1-8 in:4
- [Mate]: Bearing Mount Spacer 1-8 in:3 ↔ Bearing Mount Spacer 1-8 in:4
- [Mate]: Bearing Mount Spacer 1-8 in:3 ↔ Bearing Mount Spacer 1-8 in:4
- Mate:555: Vex Pro 1x1 rectangular tubing 14 in length:6 ↔ Bearing Mount Spacer 1-8 in:4
- Flush:15: Hex Bearing 1-2 in (FR8ZZ-Hex, am-0279):7 ↔ Hex Bearing 1-2 in (FR8ZZ-Hex, am-0279):8
- Mate:560: Hex Bearing 1-2 in (FR8ZZ-Hex, am-0279):7 ↔ Hex Shaft 1-2 in (am-0856):4
- Mate:561: Hex Bearing 1-2 in (FR8ZZ-Hex, am-0279):7 ↔ Hex Shaft 1-2 in (am-0856):4
- Mate:562: Hex Shaft 1-2 in (am-0856):4 ↔ Vex Pro 1x1 rectangular tubing 14 in length (roller):1
- Mate:563: Hex Shaft 1-2 in (am-0856):4 ↔ Vex Pro 1x1 rectangular tubing 14 in length (roller):1
- Mate:566: Vex Pro VersaPlanetary Side Mount:1 ↔ Vex Pro 1x1 rectangular tubing 14 in length (roller):1
- Mate:567 (2.3813 mm): Hex Bearing 1-2 in (FR8ZZ-Hex, am-0279):7 ↔ Vex Pro 1x1 rectangular tubing 14 in length (roller):1
- [Mate]: Bearing Mount Spacer 1-8 in:5 ↔ Bearing Mount Spacer 1-8 in:6
- [Mate]: Bearing Mount Spacer 1-8 in:5 ↔ Bearing Mount Spacer 1-8 in:6
- [Mate]: Bearing Mount Spacer 1-8 in:5 ↔ Bearing Mount Spacer 1-8 in:6
- [Mate]: Bearing Mount Spacer 1-8 in:7 ↔ Bearing Mount Spacer 1-8 in:8
- [Mate]: Bearing Mount Spacer 1-8 in:7 ↔ Bearing Mount Spacer 1-8 in:8
- [Mate]: Bearing Mount Spacer 1-8 in:7 ↔ Bearing Mount Spacer 1-8 in:8
- [Flush]: Hex Bearing 1-2 in (FR8ZZ-Hex, am-0279):9 ↔ Hex Bearing 1-2 in (FR8ZZ-Hex, am-0279):10
- [Mate]: Hex Bearing 1-2 in (FR8ZZ-Hex, am-0279):9 ↔ Hex Shaft 1-2 in (am-0856):5
- [Mate]: Hex Bearing 1-2 in (FR8ZZ-Hex, am-0279):9 ↔ Hex Shaft 1-2 in (am-0856):5
- [Mate]: Hex Shaft 1-2 in (am-0856):5 ↔ Vex Pro 1x1 rectangular tubing 14 in length (roller):2
- [Mate]: Hex Shaft 1-2 in (am-0856):5 ↔ Vex Pro 1x1 rectangular tubing 14 in length (roller):2
- [Mate] (2.3813 mm): Hex Bearing 1-2 in (FR8ZZ-Hex, am-0279):9 ↔ Vex Pro 1x1 rectangular tubing 14 in length (roller):2
- Mate:615: Vex Pro 1x1 rectangular tubing 14 in length:5 ↔ Bearing Mount Spacer 1-8 in:8
- Mate:618: Vex Pro 1x1 rectangular tubing 14 in length:5 ↔ Bearing Mount Spacer 1-8 in:6
- Flush:19 (15.0812 mm): Hex Bearing 1-2 in (FR8ZZ-Hex, am-0279):9 ↔ Hex Shaft 1-2 in (am-0856):5
- Mate:621: Vex Pro End Bearing Mount:4 ↔ Vex Pro 1x1 rectangular tubing 14 in length (roller):1
- Mate:624: Vex Pro End Bearing Mount:5 ↔ Vex Pro 1x1 rectangular tubing 14 in length (roller):1
- Mate:629: Vex Pro End Bearing Mount:8 ↔ Vex Pro 1x1 rectangular tubing 14 in length (roller):2
- Flush:20: Vex Pro 1x1 rectangular tubing 14 in length:5 ↔ Vex Pro 1x1 rectangular tubing 14 in length:6
- Mate:631: Vex Pro End Bearing Mount:7 ↔ Vex Pro 1x1 rectangular tubing 14 in length (roller):2
- Mate:632: Roller End Cap Drive (3-D Printed):5 ↔ Hex Bearing 1-2 in (FR8ZZ-Hex, am-0279):6
- Mate:633: Hex Shaft Aluminum 1-2 in (am-2291):2 ↔ Hex Shaft Collar 1-2 in (7552K500):23
- Mate:634: Hex Shaft Aluminum 1-2 in (am-2291):2 ↔ Hex Shaft Collar 1-2 in (7552K500):23
- Mate:635: Roller End Cap Drive (3-D Printed):5 ↔ Hex Shaft Collar 1-2 in (7552K500):23
- Flush:21: Vex Pro 1x1 rectangular tubing 14 in length (roller):1 ↔ Vex Pro 1x1 rectangular tubing 14 in length (roller):2
- Mate:642: Vex Pro 1x1 rectangular tubing 14 in length:6 ↔ Vex Pro 90 degree gusset:11
- Mate:650: Vex Pro 90 degree gusset:15 ↔ Vex Pro 1x1 rectangular tubing 4 in length:1
- Mate:651: Vex Pro 90 degree gusset:15 ↔ Vex Pro 1x1 rectangular tubing 4 in length:1
- Mate:652: Vex Pro 90 degree gusset:15 ↔ Vex Pro 1x1 rectangular tubing 4 in length:1
- Mate:653: Vex Pro 1x1 rectangular tubing 14 in length:5 ↔ Vex Pro 90 degree gusset:14
- Mate:654: Vex Pro 1x1 rectangular tubing 14 in length:5 ↔ Vex Pro 90 degree gusset:14
- Mate:655: Vex Pro 1x1 rectangular tubing 14 in length:5 ↔ Vex Pro 90 degree gusset:14
- Mate:656: Vex Pro 90 degree gusset:18 ↔ Vex Pro 1x1 rectangular tubing 4 in length:2
- Mate:657: Vex Pro 90 degree gusset:18 ↔ Vex Pro 1x1 rectangular tubing 4 in length:2
- Mate:658: Vex Pro 1x1 rectangular tubing 14 in length:6 ↔ Vex Pro 90 degree gusset:18
- Mate:659: Vex Pro 90 degree gusset:18 ↔ Vex Pro 1x1 rectangular tubing 4 in length:2
- Mate:660: Vex Pro 1x1 rectangular tubing 14 in length:6 ↔ Vex Pro 90 degree gusset:18
- Mate:661: Vex Pro 1x1 rectangular tubing 14 in length:6 ↔ Vex Pro 90 degree gusset:18
- Mate:666: Clamp with Piston Assembly:2 ↔ Pneumatic Piston Front Flange (Rt Custom):2
- Mate:668: Clamp with Piston Assembly:2 ↔ Pneumatic Piston Front Flange (Rt Custom):2
- Mate:669: Clamp with Piston Assembly:2 ↔ Pneumatic Piston Front Flange (Rt Custom):2
- Mate:673: Clamp with Piston Assembly:1 ↔ Pneumatic Piston Front Flange (Lt Custom):1
- Mate:683: Vex Pro 1x1 rectangular tubing 4 in length:1 ↔ Pneumatic Piston Back Flange (Rt Custom):1
- Mate:684: Vex Pro 1x1 rectangular tubing 4 in length:1 ↔ Pneumatic Piston Back Flange (Rt Custom):1
- Mate:685: Vex Pro 1x1 rectangular tubing 4 in length:1 ↔ Pneumatic Piston Back Flange (Rt Custom):1
- Mate:686: 3 Postion Pneumatic Cylinder (9-16 in Bore, .25 in,2 in stroke):1 ↔ Pneumatic Piston Back Flange (Rt Custom):1
- Mate:687: 3 Postion Pneumatic Cylinder (9-16 in Bore, .25 in,2 in stroke):1 ↔ Pneumatic Piston Back Flange (Rt Custom):1
- Mate:688: 3 Postion Pneumatic Cylinder (9-16 in Bore, .25 in,2 in stroke):1 ↔ Pneumatic Piston Back Flange (Rt Custom):1
- Mate:689: Clamp with Piston Assembly:1 ↔ Pneumatic Piston Front Flange (Lt Custom):1
- Mate:690: Clamp with Piston Assembly:1 ↔ Pneumatic Piston Front Flange (Lt Custom):1
- Mate:691: 3 Postion Pneumatic Cylinder (9-16 in Bore, .25 in,2 in stroke):1 ↔ Pneumatic Piston Front Flange (Lt Custom):1
- Mate:694: Vex Pro 1x1 rectangular tubing 4 in length:2 ↔ Pneumatic Piston Back Flange (Right Custom):1
- Mate:699: Vex Pro 1x1 rectangular tubing 4 in length:2 ↔ Pneumatic Piston Back Flange (Right Custom):1
- Mate:700: Vex Pro 1x1 rectangular tubing 4 in length:2 ↔ Pneumatic Piston Back Flange (Right Custom):1
- Mate:701: 3 Postion Pneumatic Cylinder (9-16 in Bore, .25 in,2 in stroke):2 ↔ Pneumatic Piston Back Flange (Right Custom):1
- Mate:702: 3 Postion Pneumatic Cylinder (9-16 in Bore, .25 in,2 in stroke):2 ↔ Pneumatic Piston Back Flange (Right Custom):1
- Mate:703: 3 Postion Pneumatic Cylinder (9-16 in Bore, .25 in,2 in stroke):2 ↔ Pneumatic Piston Back Flange (Right Custom):1
- Mate:704: Hex Shaft Collar 1-2 in (7552K500):21 ↔ Hex Shaft 1-2 in 5 in long (am-0856):1
- Mate:705: Hex Shaft Collar 1-2 in (7552K500):21 ↔ Hex Shaft 1-2 in 5 in long (am-0856):1
- Mate:706: Hex Shaft Collar 1-2 in (7552K500):20 ↔ Hex Shaft 1-2 in 5 in long (am-0856):1
- Mate:707: Hex Shaft Collar 1-2 in (7552K500):20 ↔ Hex Shaft 1-2 in 5 in long (am-0856):1
- Mate:708: Gusset 3 (R-L) (Custom):1 ↔ Hex Shaft 1-2 in 5 in long (am-0856):1
- Mate:709: Gusset 3 (R-L) (Custom):1 ↔ Hex Shaft 1-2 in 5 in long (am-0856):1
- Flush:22 (-3.175 mm): Hex Shaft Collar 1-2 in (7552K500):21 ↔ Hex Shaft 1-2 in 5 in long (am-0856):1
- Mate:710: Hex Shaft 1-2 in 5 in long (am-0856):1 ↔ Timing Pulley (HTD 5mm) - 18T 9mm Double Flange, 1-2 in Hex (VexPro):5
- Mate:711: Hex Shaft 1-2 in 5 in long (am-0856):1 ↔ Timing Pulley (HTD 5mm) - 18T 9mm Double Flange, 1-2 in Hex (VexPro):5
- Mate:712: Hex Shaft Collar 1-2 in (7552K500):20 ↔ Timing Pulley (HTD 5mm) - 18T 9mm Double Flange, 1-2 in Hex (VexPro):5
- Mate:713: Timing Pulley (HTD 5mm) - 18T 9mm Double Flange, 1-2 in Hex (VexPro):5 ↔ Hex Shaft Collar 1-2 in (7552K500):24
- Mate:714: Hex Shaft 1-2 in 5 in long (am-0856):1 ↔ Hex Shaft Collar 1-2 in (7552K500):24
- Mate:715: Hex Shaft 1-2 in 5 in long (am-0856):1 ↔ Hex Shaft Collar 1-2 in (7552K500):24
- Mate:726 (50.8 mm): Hex Shaft Collar 1-2 in (7552K500):20 ↔ Gusset 3 (R-L) (Custom):1
- Mate:735: Bearing Mount Spacer 1-8 in:7 ↔ Vex Pro End Bearing Mount (Bolt):1
- Mate:736: Bearing Mount Spacer 1-8 in:7 ↔ Vex Pro End Bearing Mount (Bolt):1
- Mate:737: Bearing Mount Spacer 1-8 in:7 ↔ Vex Pro End Bearing Mount (Bolt):1
- Mate:738: Hex Bearing 1-2 in (FR8ZZ-Hex, am-0279):10 ↔ Vex Pro End Bearing Mount (Bolt):1
- Mate:739: Hex Bearing 1-2 in (FR8ZZ-Hex, am-0279):10 ↔ Vex Pro End Bearing Mount (Bolt):1
- Mate:740: Bearing Mount Spacer 1-8 in:5 ↔ Vex Pro End Bearing Mount (Bolt):2
- Mate:741: Bearing Mount Spacer 1-8 in:5 ↔ Vex Pro End Bearing Mount (Bolt):2
- Mate:742: Bearing Mount Spacer 1-8 in:5 ↔ Vex Pro End Bearing Mount (Bolt):2
- Flush:23 (-9.525 mm): Hex Bearing 1-2 in (FR8ZZ-Hex, am-0279):7 ↔ Hex Shaft 1-2 in (am-0856):4
- Mate:743: Bearing Mount Spacer 1-8 in:3 ↔ Vex Pro End Bearing Mount (Bolt):3
- Mate:744: Bearing Mount Spacer 1-8 in:3 ↔ Vex Pro End Bearing Mount (Bolt):3
- Mate:745: Bearing Mount Spacer 1-8 in:3 ↔ Vex Pro End Bearing Mount (Bolt):3
- Mate:746: Hex Bearing 1-2 in (FR8ZZ-Hex, am-0279):8 ↔ Vex Pro End Bearing Mount (Bolt):3
- Mate:747: Hex Bearing 1-2 in (FR8ZZ-Hex, am-0279):8 ↔ Vex Pro End Bearing Mount (Bolt):3
- Mate:748: Bearing Mount Spacer 1-8 in:1 ↔ Vex Pro End Bearing Mount (Bolt):4
- Mate:749: Bearing Mount Spacer 1-8 in:1 ↔ Vex Pro End Bearing Mount (Bolt):4
- Mate:750: Bearing Mount Spacer 1-8 in:1 ↔ Vex Pro End Bearing Mount (Bolt):4
- Mate:751: 3 Postion Pneumatic Cylinder (9-16 in Bore, .25 in,2 in stroke):2 ↔ Pneumatic Piston Front Flange (Rt Custom):2
- Mate:752: Hex Bearing 1-2 in (FR8ZZ-Hex, am-0279):9 ↔ Vex Pro End Bearing Mount (Bolt):2
- Mate:753: Hex Bearing 1-2 in (FR8ZZ-Hex, am-0279):9 ↔ Vex Pro End Bearing Mount (Bolt):2
- Mate:754: Hex Bearing 1-2 in (FR8ZZ-Hex, am-0279):7 ↔ Vex Pro End Bearing Mount (Bolt):4
- Mate:755: Hex Bearing 1-2 in (FR8ZZ-Hex, am-0279):7 ↔ Vex Pro End Bearing Mount (Bolt):4
- Mate:758: Hex Bearing 1-2 in (FR8ZZ-Hex, am-0279):5 ↔ Hex Shaft Aluminum 1-2 in (am-2291):2
- Mate:759: Hex Bearing 1-2 in (FR8ZZ-Hex, am-0279):5 ↔ Hex Shaft Aluminum 1-2 in (am-2291):2
- Mate:760: Vex Pro End Bearing Mount:8 ↔ Vex Pro 1x1 rectangular tubing 14 in length (roller):2
- Mate:761: Vex Pro End Bearing Mount:8 ↔ Vex Pro 1x1 rectangular tubing 14 in length (roller):2
- Mate:762: Vex Pro End Bearing Mount:5 ↔ Vex Pro 1x1 rectangular tubing 14 in length (roller):1
- Mate:763: Vex Pro End Bearing Mount:5 ↔ Vex Pro 1x1 rectangular tubing 14 in length (roller):1
- Mate:764: Vex Pro End Bearing Mount:4 ↔ Vex Pro 1x1 rectangular tubing 14 in length (roller):1
- Mate:765: Vex Pro End Bearing Mount:4 ↔ Vex Pro 1x1 rectangular tubing 14 in length (roller):1
- Mate:766: Vex Pro End Bearing Mount:7 ↔ Vex Pro 1x1 rectangular tubing 14 in length (roller):2
- Mate:767: Vex Pro End Bearing Mount:7 ↔ Vex Pro 1x1 rectangular tubing 14 in length (roller):2
- Mate:774: Hex Shaft 1-2 in (am-0856):4 ↔ Hex Bearing 1-2 in (FR8ZZ-Hex, am-0279):8
- Mate:775: Hex Shaft 1-2 in (am-0856):5 ↔ Hex Bearing 1-2 in (FR8ZZ-Hex, am-0279):10
- Mate:776: Vex Pro 1x1 rectangular tubing 14 in length:6 ↔ Bearing Mount Spacer 1-8 in:2
- Mate:777: Vex Pro 1x1 rectangular tubing 14 in length:6 ↔ Bearing Mount Spacer 1-8 in:2
- Mate:778: Vex Pro 1x1 rectangular tubing 14 in length:6 ↔ Bearing Mount Spacer 1-8 in:4
- Mate:779: Vex Pro VersaPlanetary Side Mount:1 ↔ Vex Pro 1x1 rectangular tubing 14 in length (roller):1
- Mate:780: Vex Pro VersaPlanetary Side Mount:1 ↔ Vex Pro 1x1 rectangular tubing 14 in length (roller):1
- Mate:783: Vex Pro 90 degree gusset:18 ↔ Roller Piston (3 Position, .25 and 1.125 in stroke, 9-16 bore):1
- Flush:24: Vex Pro 1x1 rectangular tubing 14 in length:5 ↔ Bearing Mount Spacer 1-8 in:8
- Flush:25: Vex Pro 1x1 rectangular tubing 14 in length:5 ↔ Vex Pro End Bearing Mount (Bolt):2
- Mate:788: Vex Pro 1x1 rectangular tubing 14 in length:6 ↔ Roller Piston (3 Position, .25 and 1.125 in stroke, 9-16 bore):1
- Mate:789: Vex Pro 1x1 rectangular tubing 14 in length:6 ↔ Roller Piston (3 Position, .25 and 1.125 in stroke, 9-16 bore):1
- Angle:1 (0 deg): Vex Pro 1x1 rectangular tubing 14 in length (roller):1 ↔ Roller Piston (3 Position, .25 and 1.125 in stroke, 9-16 bore):1
## Named parameters: d216_d210 = 0 mm, d217_d213 = 0 mm, d240_d195 = 0 mm, d241_d196 = 0 mm, d242_d197 = 0 mm, d243_d198 = 0 mm, d305_d302 = 0 mm, d306_d303 = 0 mm, d307_d304 = 0 mm, d334_d317 = 0 mm, d335_d318 = -19.05 mm, d336_d325 = 0 mm, d339_d304 = 0 mm, d343_d308 = 0 mm, d344_d309 = 0 mm, d345_d310 = 0 mm, d346_d316 = 0 mm, d347_d326 = 0 mm, d348_d327 = -9.525 mm, d349_d328 = 0 mm, d350_d329 = 0 mm, d351_d330 = 0 mm, d352_d331 = 0 mm, d353_d332 = 0 mm, d354_d333 = 0 mm, d175_d158 = 0 mm, d176_d159 = 0 mm, d177_d160 = 0 mm, d729_d175_d158 = 0 mm, d730_d176_d159 = 0 mm, d731_d177_d160 = 0 mm, d764_d175_d158 = 0 mm, d765_d176_d159 = 0 mm, d766_d177_d160 = 0 mm, d770_d743 = 0 mm, d771_d744 = 0 mm, d772_d745 = 0 mm, d773_d746 = 0 mm, d774_d750 = 2.38125 mm, d781_d729_d175_d158 = 0 mm, d782_d730_d176_d159 = 0 mm, d783_d731_d177_d160 = 0 mm, d791_d742 = 0 mm
